# Autodesk Inventor assembly: motor_bell_ccwprop
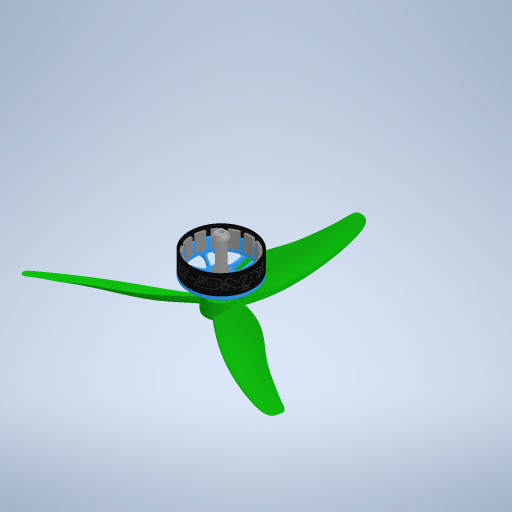
[picture p0: Inventor's stored thumbnail of the model, 512x512]
Saved by Autodesk Inventor 2024 (Build 280153000, 153)
## iProperties
Created: 2024-03-08
Part Number: motor_bell_ccwprop
Document SubType Name: Assembly
Designer: nicoe
Sending System: Creo  TM  7.0
Author: nicoe
## Documents named in this file (7)
- D:\users\nicoe\OneDrive\OneDrive - Stellenbosch University\Desktop\Nico_Masters\1. Drone Constrution\CAD Files\iflight xing-e 2306(To replace R5)\Broken up motor\motor_bell_ccwprop.iam
- D:\users\nicoe\OneDrive\OneDrive - Stellenbosch University\Desktop\Nico_Masters\1. Drone Constrution\CAD Files\iflight xing-e 2306(To replace R5)\motor xing\cely_motor\MOTOR_VRCH1.ipt
- D:\users\nicoe\OneDrive\OneDrive - Stellenbosch University\Desktop\Nico_Masters\1. Drone Constrution\CAD Files\iflight xing-e 2306(To replace R5)\motor xing\cely_motor\MOTOR_VRCH.ipt
- D:\users\nicoe\OneDrive\OneDrive - Stellenbosch University\Desktop\Nico_Masters\1. Drone Constrution\CAD Files\iflight xing-e 2306(To replace R5)\motor xing\cely_motor\MOTOR_VRCH2.ipt
- D:\users\nicoe\OneDrive\OneDrive - Stellenbosch University\Desktop\Nico_Masters\1. Drone Constrution\CAD Files\iflight xing-e 2306(To replace R5)\motor xing\cely_motor\MOTOR_MAGNET.ipt
- D:\users\nicoe\OneDrive\OneDrive - Stellenbosch University\Desktop\Nico_Masters\1. Drone Constrution\CAD Files\iflight xing-e 2306(To replace R5)\motor xing\cely_motor\MOTOR_SKRUTKA.ipt
- D:\users\nicoe\OneDrive\OneDrive - Stellenbosch University\Desktop\Nico_Masters\1. Drone Constrution\CAD Files\Gemfan Hurricane 51466\Gemfan Hurricane 51466\[CCW] Gemfan Hurricane 51466.iam
## Components (6 placed, 6 different names)
1. MOTOR_VRCH1
2. MOTOR_VRCH — Mate:1, Flush:1
3. MOTOR_VRCH2
4. MOTOR_MAGNET
5. MOTOR_SKRUTKA
6. [CCW] Gemfan Hurricane 51466:1 [sub-assembly] — Mate:1, Flush:1, Mate:2
## Relationships (3: Mate 2, Flush 1)
- Mate:1: MOTOR_VRCH ↔ [CCW] Gemfan Hurricane 51466:1
- Flush:1 (3 mm): MOTOR_VRCH ↔ [CCW] Gemfan Hurricane 51466:1
- Mate:2: [CCW] Gemfan Hurricane 51466:1
